# Autodesk Inventor assembly: plate_assembly
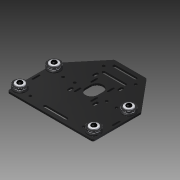
[picture p0: Inventor's stored thumbnail of the model, 180x180]
Saved by Autodesk Inventor 2014 (Build 180170000, 170)
## iProperties
Created: 2013-05-29
Part Number: plate_assembly
Document SubType Name: Assembly
Designer: Edward
Author: Edward
## Documents named in this file (7)
- C:\Users\Edward\Desktop\Shapeoko_v2.0\plate_assembly.iam
- C:\Users\Edward\Desktop\Shapeoko_v2.0\S2_mm.ipt
- C:\Users\Edward\Desktop\Shapeoko_v2.0\B18033.ipt
- C:\Users\Edward\Desktop\Shapeoko_v2.0\B30037.iam
- C:\Users\Edward\Desktop\Shapeoko_v2.0\91239A233.ipt
- C:\Users\Edward\Desktop\Shapeoko_v2.0\SM-H03.ipt
- C:\Users\Edward\Desktop\Shapeoko_v2.0\SM-H04.ipt
## Components (19 placed, 6 different names)
1. S2_mm:1 — Insert:3, Insert:5, Insert:9, Mate:2, Insert:10, Mate:4, Insert:15, Insert:16
2. B18033:1 — Insert:10, Mate:3
3. B18033:2 — Mate:1, Insert:9
4. B30037:4 [sub-assembly] — Insert:2, Insert:4
5. SM-H03:1 — Insert:2, Insert:3
6. 91239A233:2 — Insert:4
7. SM-H03:2 — Insert:11, Mate:4
8. SM-H04:2 — Insert:6
9. SM-H03:4 — Insert:16, Insert:17
10. SM-H03:5 — Insert:14, Insert:15
11. SM-H03:6 — Insert:7, Mate:2
12. SM-H03:7 — Insert:5, Insert:6
13. 91239A233:3 — Insert:8, Mate:1
14. B30037:5 [sub-assembly] — Insert:7, Insert:8
15. 91239A233:4 — Insert:12, Mate:3
16. B30037:6 [sub-assembly] — Insert:11, Insert:12
17. 91239A233:5 — Insert:13
18. B30037:7 [sub-assembly] — Insert:13, Insert:14
19. SM-H04:3 — Insert:17
## Relationships (20: Insert 16, Mate 4)
- Insert:2: B30037:4 ↔ SM-H03:1
- Insert:3: S2_mm:1 ↔ SM-H03:1
- Insert:4: B30037:4 ↔ 91239A233:2
- Insert:5: S2_mm:1 ↔ SM-H03:7
- Insert:6: SM-H04:2 ↔ SM-H03:7
- Insert:7: SM-H03:6 ↔ B30037:5
- Insert:8: 91239A233:3 ↔ B30037:5
- Mate:1: B18033:2 ↔ 91239A233:3
- Insert:9: S2_mm:1 ↔ B18033:2
- Mate:2: S2_mm:1 ↔ SM-H03:6
- Insert:10: S2_mm:1 ↔ B18033:1
- Insert:11: SM-H03:2 ↔ B30037:6
- Insert:12: 91239A233:4 ↔ B30037:6
- Mate:3: B18033:1 ↔ 91239A233:4
- Mate:4: S2_mm:1 ↔ SM-H03:2
- Insert:13: 91239A233:5 ↔ B30037:7
- Insert:14: SM-H03:5 ↔ B30037:7
- Insert:15: S2_mm:1 ↔ SM-H03:5
- Insert:16: S2_mm:1 ↔ SM-H03:4
- Insert:17: SM-H03:4 ↔ SM-H04:3
